# Autodesk Inventor assembly: Assembly1
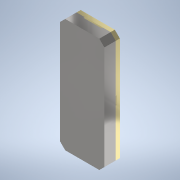
[picture p0: Inventor's stored thumbnail of the model, 180x180]
Saved by Autodesk Inventor 2022 (Build 260153000, 153)
## iProperties
Created: 2022-05-30
Part Number: Assembly1
Document SubType Name: Assembly
Designer: Aakif
Author: Aakif
## Documents named in this file (3)
- D:\proyek pribadi\nata\Assembly1.iam
- D:\proyek pribadi\nata\enclosed base.ipt
- D:\proyek pribadi\nata\enclosed top.ipt
## Components (2 placed, 2 different names)
1. enclosed top:1 — Mate:1
2. enclosed base:1 — Mate:1
## Relationships (1: Mate 1)
- Mate:1: enclosed top:1 ↔ enclosed base:1
